# Autodesk Inventor assembly: RobotStandAssy
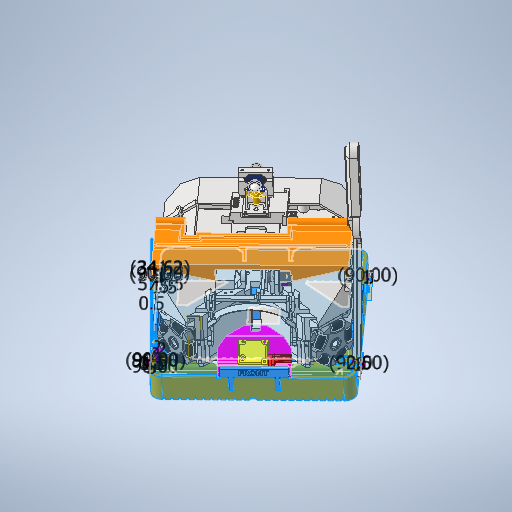
[picture p0: Inventor's stored thumbnail of the model, 512x512]
Saved by Autodesk Inventor 2025.1 (Build 291241000, 241)
## iProperties
Created: 2026-05-10
Part Number: RobotStandAssy
Document SubType Name: Assembly
Designer: User
Author: User
## Documents named in this file (11)
- D:\One Drive\OneDrive - Politeknik Sultan Salahuddin Abdul Aziz Shah\Documents\Inventor\RobosotPSA\RobotStandAssy.iam
- D:\One Drive\OneDrive - Politeknik Sultan Salahuddin Abdul Aziz Shah\Documents\Inventor\RobosotPSA\HalfRobotAssy.iam
- D:\One Drive\OneDrive - Politeknik Sultan Salahuddin Abdul Aziz Shah\Documents\Inventor\RobosotPSA\RobotStand.ipt
- D:\One Drive\OneDrive - Politeknik Sultan Salahuddin Abdul Aziz Shah\Documents\Inventor\RobosotPSA\RobotStandBase.ipt
- D:\One Drive\OneDrive - Politeknik Sultan Salahuddin Abdul Aziz Shah\Documents\Inventor\RobosotPSA\FrontLock.ipt
- D:\One Drive\OneDrive - Politeknik Sultan Salahuddin Abdul Aziz Shah\Documents\Inventor\RobosotPSA\LatchLock.ipt
- D:\One Drive\OneDrive - Politeknik Sultan Salahuddin Abdul Aziz Shah\Documents\Inventor\RobosotPSA\LatchCover.ipt
- D:\One Drive\OneDrive - Politeknik Sultan Salahuddin Abdul Aziz Shah\Documents\Inventor\RobosotPSA\BaseShaft.ipt
- D:\One Drive\OneDrive - Politeknik Sultan Salahuddin Abdul Aziz Shah\Documents\Inventor\RobosotPSA\RobotStandHandle.ipt
- D:\One Drive\OneDrive - Politeknik Sultan Salahuddin Abdul Aziz Shah\Documents\Inventor\RobosotPSA\TheHandle.ipt
- D:\One Drive\OneDrive - Politeknik Sultan Salahuddin Abdul Aziz Shah\Documents\Inventor\RobosotPSA\TheHandle_Left.ipt
## Components (12 placed, 10 different names)
1. HalfRobotAssy:1 [sub-assembly] — Mate:1, Flush:8
2. RobotStand:1 — Mate:1, Mate:3, Flush:2, Flush:3
3. HalfRobotAssy:2 [sub-assembly] — Mate:3
4. RobotStandBase:1 — Flush:2, Flush:6, Flush:7
5. FrontLock:1 — Flush:3, Flush:4, Flush:5
6. LatchLock:1 — Flush:4
7. LatchCover:1 — Flush:5
8. BaseShaft:1 — Flush:6, Flush:7
9. BaseShaft:2
10. RobotStandHandle:1 — Flush:9, Flush:10
11. TheHandle:1
12. TheHandle_Left:1
## Relationships (11: Flush 9, Mate 2)
- Mate:1: HalfRobotAssy:1 ↔ RobotStand:1
- Mate:3 (-25 mm): RobotStand:1 ↔ HalfRobotAssy:2
- Flush:2: RobotStand:1 ↔ RobotStandBase:1
- Flush:3: RobotStand:1 ↔ FrontLock:1
- Flush:4: FrontLock:1 ↔ LatchLock:1
- Flush:5: FrontLock:1 ↔ LatchCover:1
- Flush:6: RobotStandBase:1 ↔ BaseShaft:1
- Flush:7: RobotStandBase:1 ↔ BaseShaft:1
- Flush:8 (1 mm): HalfRobotAssy:1
- Flush:9: RobotStandHandle:1
- Flush:10: RobotStandHandle:1
